# Autodesk Inventor assembly: Assembly_Insert_Lens_mount_fixed
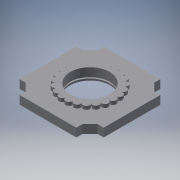
[picture p0: Inventor's stored thumbnail of the model, 180x180]
Saved by Autodesk Inventor 2019 (Build 230136000, 136)
## iProperties
Created: 2019-10-23
Part Number: Assembly_Insert_Lens_mount_fixed
Document SubType Name: Assembly
Designer: marsikovabarbora
Author: marsikovabarbora
## Documents named in this file (3)
- C:\Users\marsikovabarbora\Documents\GitHub\UC2-GIT\CAD\ASSEMBLY_CUBE_Lens_v2\STL\Lens_Insert\Assembly_Insert_Lens_mount_fixed.iam
- C:\Users\marsikovabarbora\Documents\GitHub\UC2-GIT\CAD\ASSEMBLY_CUBE_Lens_v2\STL\Lens_Insert\20_Lens_holder.ipt
- C:\Users\marsikovabarbora\Documents\GitHub\UC2-GIT\CAD\ASSEMBLY_CUBE_Lens_v2\STL\Lens_Insert\20_Lens_holder_clamp.ipt
## Components (2 placed, 2 different names)
1. 20_Lens_holder:1 — Flush:1
2. 20_Lens_holder_clamp:1 — Flush:1
## Relationships (1: Flush 1)
- Flush:1: 20_Lens_holder:1 ↔ 20_Lens_holder_clamp:1
